# Autodesk Inventor assembly: 123
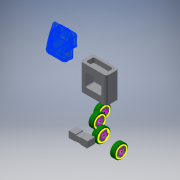
[picture p0: Inventor's stored thumbnail of the model, 180x180]
Saved by Autodesk Inventor 2018 (Build 220112000, 112)
## iProperties
Created: 2019-04-04
Part Number: 123
Document SubType Name: Assembly
Designer: This kid
Author: This kid
## Documents named in this file (7)
- C:\Users\10043883\Documents\GitHub\IED-files\123.iam
- C:\Users\10043883\Documents\GitHub\IED-files\5.5\5.5a\ARTHURW5.5a AXLE.ipt
- C:\Users\10043883\Documents\GitHub\IED-files\5.5\5.5a\AWAutomobloxTire.ipt
- C:\Users\10043883\Documents\GitHub\IED-files\5.5\5.5b\ARTHURw5.5bAutomobloxConnectorPiece.ipt
- C:\Users\10043883\Documents\GitHub\IED-files\5.2\5.2b\AW5.2bWINDSHIELD.ipt
- C:\Users\10043883\Documents\GitHub\IED-files\5.2\5.2b\AutomobloxWheel.ipt
- C:\Users\10043883\Desktop\T9 Passenger Section (1).ipt
## Components (18 placed, 6 different names)
1. ARTHURW5.5a AXLE:1 — Mate:1
2. AWAutomobloxTire:1 — Mate:2
3. ARTHURw5.5bAutomobloxConnectorPiece:1
4. AW5.2bWINDSHIELD:1
5. AutomobloxWheel:1 — Mate:1, Mate:2
6. ARTHURW5.5a AXLE:2
7. AWAutomobloxTire:2
8. AutomobloxWheel:2
9. ARTHURW5.5a AXLE:3
10. AWAutomobloxTire:3
11. AutomobloxWheel:3
12. ARTHURW5.5a AXLE:4
13. AWAutomobloxTire:4
14. AutomobloxWheel:4
15. ARTHURW5.5a AXLE:5
16. AWAutomobloxTire:5
17. AutomobloxWheel:5
18. T9 Passenger Section (1):1
## Relationships (10: Mate 10)
- Mate:1: ARTHURW5.5a AXLE:1 ↔ AutomobloxWheel:1
- Mate:2: AWAutomobloxTire:1 ↔ AutomobloxWheel:1
- [Mate]: ARTHURW5.5a AXLE:2 ↔ AutomobloxWheel:2
- [Mate]: AWAutomobloxTire:2 ↔ AutomobloxWheel:2
- [Mate]: ARTHURW5.5a AXLE:3 ↔ AutomobloxWheel:3
- [Mate]: AWAutomobloxTire:3 ↔ AutomobloxWheel:3
- [Mate]: ARTHURW5.5a AXLE:4 ↔ AutomobloxWheel:4
- [Mate]: AWAutomobloxTire:4 ↔ AutomobloxWheel:4
- [Mate]: ARTHURW5.5a AXLE:5 ↔ AutomobloxWheel:5
- [Mate]: AWAutomobloxTire:5 ↔ AutomobloxWheel:5
## Named parameters: d2_d0 = 0 mm, d3_d1 = 0 mm, d4_d0 = 0 mm, d5_d1 = 0 mm, d6_d0 = 0 mm, d7_d1 = 0 mm, d8_d0 = 0 mm, d9_d1 = 0 mm
